# Autodesk Inventor assembly: LegAssembly
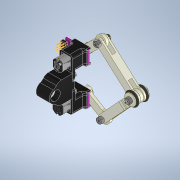
[picture p0: Inventor's stored thumbnail of the model, 180x180]
Saved by Autodesk Inventor 2022 (Build 260153000, 153)
## iProperties
Created: 2021-12-08
Part Number: LegAssembly
Document SubType Name: Assembly
Designer: JK
Author: JK
## Documents named in this file (15)
- C:\Users\JK\Documents\Inventor\N20 Leg Actuator\N20-Leg-Actuator\CADfiles\N20 Leg\LegAssembly.iam
- C:\Users\JK\Documents\Inventor\N20 Leg Actuator\N20-Leg-Actuator\CADfiles\N20Module\N20Module.iam
- C:\Users\JK\Documents\Inventor\N20 Leg Actuator\N20-Leg-Actuator\CADfiles\N20 Leg\683zz.ipt
- C:\Users\JK\Documents\Inventor\N20 Leg Actuator\N20-Leg-Actuator\CADfiles\N20 Leg\LinkB.ipt
- C:\Users\JK\Documents\Inventor\N20 Leg Actuator\N20-Leg-Actuator\CADfiles\N20 Leg\LinkA.ipt
- C:\Users\JK\Documents\Inventor\N20 Leg Actuator\N20-Leg-Actuator\CADfiles\N20 Leg\M3x12SocketBolt.ipt
- C:\Users\JK\Documents\Inventor\N20 Leg Actuator\N20-Leg-Actuator\CADfiles\N20 Leg\M3 Locknut.ipt
- C:\Users\JK\Documents\Inventor\N20 Leg Actuator\N20-Leg-Actuator\CADfiles\N20 Leg\Motorlink.ipt
- C:\Users\JK\Documents\Inventor\N20 Leg Actuator\N20-Leg-Actuator\CADfiles\N20Module\N20Module_MIR.iam
- C:\Users\JK\Documents\Inventor\N20 Leg Actuator\N20-Leg-Actuator\CADfiles\N20 Leg\MiddleJoint.ipt
- C:\Users\JK\Documents\Inventor\N20 Leg Actuator\N20-Leg-Actuator\CADfiles\N20 Leg\RubberSupport.ipt
- C:\Users\JK\Documents\Inventor\N20 Leg Actuator\N20-Leg-Actuator\CADfiles\N20 Leg\M3x20SocketBolt.ipt
- C:\Users\JK\Documents\Inventor\N20 Leg Actuator\N20-Leg-Actuator\CADfiles\N20 Leg\M3x6SocketBolt.ipt
- C:\Users\JK\Documents\Inventor\N20 Leg Actuator\N20-Leg-Actuator\CADfiles\N20 Leg\9mmSpacer.ipt
- C:\Users\JK\Documents\Inventor\N20 Leg Actuator\N20-Leg-Actuator\CADfiles\N20 Leg\oring.ipt
## Components (25 placed, 14 different names)
1. 683zz:1 — Coincidencia:10, Coincidencia:11, Coincidencia:36
2. 683zz:2 — Coincidencia:13, Coincidencia:14, Coincidencia:35
3. LinkB:1 — Coincidencia:10, Coincidencia:11, Coincidencia:12, Nivelación:4, Coincidencia:24, Coincidencia:28, Coincidencia:34, Nivelación:6
4. 683zz:3 — Coincidencia:12, Nivelación:4, Coincidencia:15, Coincidencia:21
5. LinkA:1 — Coincidencia:13, Coincidencia:14, Coincidencia:15, Coincidencia:21, Coincidencia:23, Coincidencia:27, Coincidencia:33, Coincidencia:44, Coincidencia:45, Coincidencia:46, Coincidencia:47, Nivelación:13, Coincidencia:60
6. M3x12SocketBolt:1 — Coincidencia:24, Coincidencia:28, Coincidencia:29
7. M3x12SocketBolt:2 — Coincidencia:23, Coincidencia:27, Coincidencia:30
8. M3 Locknut:1 — Coincidencia:29, Coincidencia:34
9. M3 Locknut:2 — Coincidencia:30, Coincidencia:33
10. M3 Locknut:3 — Coincidencia:48, Coincidencia:49
11. Motorlink:1 — Coincidencia:36, Nivelación:5, Nivelación:6, Coincidencia:40, Nivelación:8
12. Motorlink:2 — Coincidencia:35, Nivelación:5, Coincidencia:37, Nivelación:7
13. N20Module:1 [sub-assembly] — Coincidencia:37, Coincidencia:38, Nivelación:7, Coincidencia:41, Coincidencia:43, Coincidencia:54, Coincidencia:55
14. N20Module_MIR:1 [sub-assembly] — Coincidencia:39, Coincidencia:40, Nivelación:8, Coincidencia:42, Coincidencia:52, Coincidencia:53
15. MiddleJoint:1 — Coincidencia:41, Coincidencia:42, Coincidencia:43, Coincidencia:57, Nivelación:12
16. RubberSupport:1 — Coincidencia:46, Coincidencia:47, Coincidencia:48, Coincidencia:49, Coincidencia:59
17. RubberSupport:2 — Coincidencia:44, Coincidencia:45, Coincidencia:50, Coincidencia:51, Coincidencia:58
18. M3x20SocketBolt:1 — Coincidencia:50, Coincidencia:51
19. M3x6SocketBolt:1 — Coincidencia:52, Nivelación:10, Nivelación:11
20. M3x6SocketBolt:2 — Coincidencia:53, Nivelación:11
21. M3x6SocketBolt:3 — Coincidencia:54, Nivelación:9, Nivelación:10
22. M3x6SocketBolt:4 — Coincidencia:55, Nivelación:9
23. 9mmSpacer:1 — Coincidencia:57, Nivelación:12
24. oring:1 — Coincidencia:58, Nivelación:13
25. oring:2 — Coincidencia:59, Coincidencia:60
## Relationships (50: Mate 40, Flush 10)
- Coincidencia:10 [Mate]: 683zz:1 ↔ LinkB:1
- Coincidencia:11 [Mate] (0.1 mm): 683zz:1 ↔ LinkB:1
- Coincidencia:12 [Mate]: LinkB:1 ↔ 683zz:3
- Nivelación:4 [Flush]: LinkB:1 ↔ 683zz:3
- Coincidencia:13 [Mate]: 683zz:2 ↔ LinkA:1
- Coincidencia:14 [Mate] (0.1 mm): 683zz:2 ↔ LinkA:1
- Coincidencia:15 [Mate]: 683zz:3 ↔ LinkA:1
- Coincidencia:21 [Mate]: 683zz:3 ↔ LinkA:1
- Coincidencia:23 [Mate]: LinkA:1 ↔ M3x12SocketBolt:2
- Coincidencia:24 [Mate]: LinkB:1 ↔ M3x12SocketBolt:1
- Coincidencia:27 [Mate]: LinkA:1 ↔ M3x12SocketBolt:2
- Coincidencia:28 [Mate]: LinkB:1 ↔ M3x12SocketBolt:1
- Coincidencia:29 [Mate]: M3x12SocketBolt:1 ↔ M3 Locknut:1
- Coincidencia:30 [Mate]: M3x12SocketBolt:2 ↔ M3 Locknut:2
- Coincidencia:33 [Mate]: LinkA:1 ↔ M3 Locknut:2
- Coincidencia:34 [Mate]: LinkB:1 ↔ M3 Locknut:1
- Coincidencia:35 [Mate]: 683zz:2 ↔ Motorlink:2
- Coincidencia:36 [Mate]: 683zz:1 ↔ Motorlink:1
- Nivelación:5 [Flush]: Motorlink:1 ↔ Motorlink:2
- Nivelación:6 [Flush]: LinkB:1 ↔ Motorlink:1
- Coincidencia:37 [Mate]: Motorlink:2 ↔ N20Module:1
- Coincidencia:38 [Mate]: N20Module:1
- Nivelación:7 [Flush]: Motorlink:2 ↔ N20Module:1
- Coincidencia:39 [Mate]: N20Module_MIR:1
- Coincidencia:40 [Mate]: Motorlink:1 ↔ N20Module_MIR:1
- Nivelación:8 [Flush]: Motorlink:1 ↔ N20Module_MIR:1
- Coincidencia:41 [Mate]: N20Module:1 ↔ MiddleJoint:1
- Coincidencia:42 [Mate]: N20Module_MIR:1 ↔ MiddleJoint:1
- Coincidencia:43 [Mate]: N20Module:1 ↔ MiddleJoint:1
- Coincidencia:44 [Mate]: LinkA:1 ↔ RubberSupport:2
- Coincidencia:45 [Mate]: LinkA:1 ↔ RubberSupport:2
- Coincidencia:46 [Mate]: LinkA:1 ↔ RubberSupport:1
- Coincidencia:47 [Mate]: LinkA:1 ↔ RubberSupport:1
- Coincidencia:48 [Mate]: M3 Locknut:3 ↔ RubberSupport:1
- Coincidencia:49 [Mate]: M3 Locknut:3 ↔ RubberSupport:1
- Coincidencia:50 [Mate]: RubberSupport:2 ↔ M3x20SocketBolt:1
- Coincidencia:51 [Mate]: RubberSupport:2 ↔ M3x20SocketBolt:1
- Coincidencia:52 [Mate]: N20Module_MIR:1 ↔ M3x6SocketBolt:1
- Coincidencia:53 [Mate]: N20Module_MIR:1 ↔ M3x6SocketBolt:2
- Coincidencia:54 [Mate]: N20Module:1 ↔ M3x6SocketBolt:3
- Coincidencia:55 [Mate]: N20Module:1 ↔ M3x6SocketBolt:4
- Nivelación:9 [Flush]: M3x6SocketBolt:3 ↔ M3x6SocketBolt:4
- Nivelación:10 [Flush]: M3x6SocketBolt:1 ↔ M3x6SocketBolt:3
- Nivelación:11 [Flush]: M3x6SocketBolt:1 ↔ M3x6SocketBolt:2
- Coincidencia:57 [Mate]: MiddleJoint:1 ↔ 9mmSpacer:1
- Nivelación:12 [Flush]: MiddleJoint:1 ↔ 9mmSpacer:1
- Coincidencia:58 [Mate]: RubberSupport:2 ↔ oring:1
- Coincidencia:59 [Mate]: RubberSupport:1 ↔ oring:2
- Nivelación:13 [Flush] (-1.25 mm): LinkA:1 ↔ oring:1
- Coincidencia:60 [Mate] (1.25 mm): LinkA:1 ↔ oring:2
